# Autodesk Inventor assembly: BaseAssembly
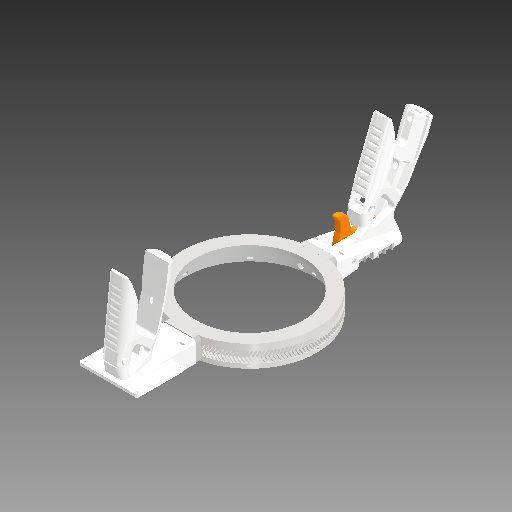
[picture p0: Inventor's stored thumbnail of the model, 512x512]
Saved by Autodesk Inventor 2020 (Build 240168000, 168)
## iProperties
Created: 2020-09-17
Part Number: BaseAssembly
Document SubType Name: Assembly
Designer: DDeGo
Author: DDeGo
## Documents named in this file (4)
- C:\Users\DDeGo\Documents\Drew\Projects\Nerf_Aimbot\Cad\BaseAssembly.iam
- C:\Users\DDeGo\Documents\Drew\Projects\Nerf_Aimbot\Cad\144 Tooth Herringbone Gear Base Mount.ipt
- C:\Users\DDeGo\Documents\Drew\Projects\Nerf_Aimbot\Cad\GripFront.ipt
- C:\Users\DDeGo\Documents\Drew\Projects\Nerf_Aimbot\ESPER\GripE.iam
## Components (3 placed, 3 different names)
1. 144 Tooth Herringbone Gear Base Mount:1 — Mate:1, Mate:2, Mate:3, Mate:4, Mate:5, Mate:6
2. GripFront:1 — Mate:2, Mate:5, Mate:6
3. GripE:1 [sub-assembly] — Mate:1, Mate:3, Mate:4
## Relationships (6: Mate 6)
- Mate:1: 144 Tooth Herringbone Gear Base Mount:1 ↔ GripE:1
- Mate:2: 144 Tooth Herringbone Gear Base Mount:1 ↔ GripFront:1
- Mate:3: 144 Tooth Herringbone Gear Base Mount:1 ↔ GripE:1
- Mate:4: 144 Tooth Herringbone Gear Base Mount:1 ↔ GripE:1
- Mate:5: 144 Tooth Herringbone Gear Base Mount:1 ↔ GripFront:1
- Mate:6: 144 Tooth Herringbone Gear Base Mount:1 ↔ GripFront:1
